# Autodesk Inventor assembly: Deck
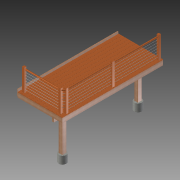
[picture p0: Inventor's stored thumbnail of the model, 180x180]
Saved by Autodesk Inventor 2015 (Build 190159000, 159)
## iProperties
Created: 2014-05-27
Part Number: Deck
Document SubType Name: Assembly
Designer: Haden
Mass: 751429 g
Surface Area: 376936 cm^2
Volume: 644413 cm^3
Density: 1.16607 g/cm^3
Author: Haden
## Documents named in this file (22)
- C:\Users\Haden\Desktop\Deck\Deck.iam
- C:\Users\Haden\Desktop\Deck\Footing.ipt
- C:\Users\Haden\Desktop\Deck\Ledger Board.ipt
- C:\Users\Haden\Desktop\Deck\Left End Board.ipt
- C:\Users\Haden\Desktop\Deck\Joist.ipt
- C:\Users\Haden\Desktop\Deck\Truss.ipt
- C:\Users\Haden\Desktop\Deck\TimberTech.ipt
- C:\Users\Haden\Desktop\Deck\Left Post.ipt
- C:\Users\Haden\Desktop\Deck\Right Post.ipt
- C:\Users\Haden\Desktop\Deck\TimberTech Post.ipt
- C:\Users\Haden\Desktop\Deck\Front Railing.ipt
- C:\Users\Haden\Desktop\Deck\Side Railing.ipt
- C:\Users\Haden\Desktop\Deck\Left Cable.ipt
- C:\Users\Haden\Desktop\Deck\Front Cable.ipt
- C:\Users\Haden\Desktop\Deck\corner cable.ipt
- C:\Users\Haden\Desktop\Deck\Corner Railing.ipt
- C:\Users\Haden\Desktop\Deck\Deck\AIP\FEA\b2f62dg5c.fins
- C:\Users\Haden\Desktop\Deck\Deck\AIP\FEA\b2f62dg5c.fsat
- C:\Users\Haden\Desktop\Deck\Deck\AIP\FEA\b2f62dg5c.ftes
- C:\Users\Haden\Desktop\Deck\Deck\AIP\FEA\b2f62dg5c.fwiz
- C:\Users\Haden\Desktop\Deck\Deck\AIP\FEA\b2f62dh28.fmsh
- C:\Users\Haden\Desktop\Deck\Deck\AIP\FEA\b2f62dh29.fres
## Components (49 placed, 15 different names)
1. Ledger Board:1 — Mate:1, Mate:3, Flush:2, Mate:7, Mate:8, Mate:9, Mate:10, Mate:11, Mate:12, Mate:13, Mate:14, Mate:15, Mate:16, Mate:17, Mate:18, Mate:19, Flush:55, Mate:21, Flush:65, Mate:51
2. Left End Board:1 — Mate:1, Flush:65, Flush:1, Flush:6, Mate:6, Flush:7, Flush:8, Mate:37, Mate:38
3. Truss:1 — Mate:4, Flush:4, Flush:5
4. Truss:2 — Mate:4, Flush:4, Flush:5, Flush:6, Mate:5, Mate:37, Mate:39, Flush:69, Flush:70
5. Truss:3 — Mate:6, Flush:7, Flush:8, Flush:78, Mate:47
6. Joist:1 — Mate:3, Flush:1, Flush:2, Mate:38, Mate:5, Flush:9, Flush:22, Mate:20, Mate:48
7. Joist:2 — Flush:9, Flush:10, Flush:22, Flush:23, Mate:7
8. Joist:3 — Flush:10, Flush:11, Flush:23, Flush:24, Mate:8
9. Joist:4 — Flush:11, Flush:12, Flush:24, Flush:25, Mate:9
10. Joist:5 — Flush:12, Flush:13, Flush:25, Flush:26, Mate:10
11. Joist:6 — Flush:13, Flush:14, Flush:26, Flush:27, Mate:11
12. Joist:7 — Flush:14, Flush:15, Flush:27, Flush:28, Mate:12
13. Joist:8 — Flush:15, Flush:16, Flush:28, Flush:29, Mate:13
14. Joist:9 — Flush:16, Flush:17, Flush:29, Flush:30, Mate:14
15. Joist:10 — Flush:17, Flush:18, Flush:30, Flush:31, Mate:15
16. Joist:11 — Flush:18, Flush:19, Flush:31, Flush:32, Mate:16
17. Joist:12 — Flush:19, Flush:20, Flush:32, Flush:33, Mate:17
18. Joist:13 — Flush:20, Flush:21, Flush:33, Flush:34, Mate:18
19. Joist:14 — Flush:21, Flush:34, Mate:19
20. TimberTech:1 — Flush:35, Flush:45, Mate:20, Flush:55, Mate:21, Mate:22
21. TimberTech:2 — Flush:35, Flush:36, Flush:45, Flush:46, Mate:22, Mate:23, Mate:61
22. TimberTech:3 — Flush:36, Flush:37, Flush:46, Flush:47, Mate:23, Mate:24
23. TimberTech:4 — Flush:37, Flush:38, Flush:47, Flush:48, Mate:24, Mate:25
24. TimberTech:5 — Flush:38, Flush:39, Flush:48, Flush:49, Mate:25, Mate:26
25. TimberTech:6 — Flush:39, Flush:40, Flush:49, Flush:50, Mate:26, Mate:27
26. TimberTech:7 — Flush:40, Flush:41, Flush:50, Flush:51, Mate:27, Mate:28
27. TimberTech:8 — Flush:41, Flush:42, Flush:51, Flush:52, Mate:28, Mate:29
28. TimberTech:9 — Flush:42, Flush:43, Flush:52, Flush:53, Mate:29, Mate:30
29. TimberTech:10 — Flush:43, Flush:44, Flush:53, Flush:54, Mate:30, Mate:31
30. TimberTech:11 — Flush:44, Flush:54, Mate:31, Flush:56, Flush:57, Mate:32
31. TimberTech:12 — Flush:56, Flush:57, Mate:32, Mate:68, Mate:71, Flush:86, Flush:87, Mate:74
32. TimberTech:13 — Flush:86, Flush:87, Mate:74
33. Footing:1 — Mate:40, Rotation:1, Rotation:2, Mate:43
34. Footing:2 — Mate:41, Rotation:1, Mate:42
35. Left Post:1 — Flush:66, Flush:67, Mate:39, Mate:40, Rotation:2, Mate:43, Flush:68, Flush:69, Flush:70
36. Right Post:1 — Flush:66, Flush:67, Mate:41, Mate:42, Flush:68
37. TimberTech Post:1 — Flush:71, Flush:74, Mate:49, Mate:50, Flush:80, Mate:55, Mate:70, Mate:73
38. TimberTech Post:2 — Flush:71, Flush:74, Flush:75, Mate:48, Mate:51, Mate:52, Flush:83, Mate:58
39. TimberTech Post:3 — Flush:75, Flush:76, Mate:45, Flush:78, Flush:79, Mate:47, Mate:49, Mate:50, Mate:53, Mate:57, Flush:84, Mate:62, Mate:69, Mate:72
40. TimberTech Post:4 — Flush:73, Flush:76, Flush:77, Mate:44, Mate:45, Flush:79, Mate:54, Mate:63
41. TimberTech Post:5 — Flush:73, Flush:77, Mate:44
42. Front Railing:1 — Mate:53, Flush:81, Flush:82, Mate:56, Mate:57
43. Front Railing:2 — Mate:54, Flush:82, Mate:56
44. Side Railing:1 — Mate:52, Flush:80, Mate:55, Flush:81, Flush:85
45. Left Cable:1 — Mate:58, Mate:59, Mate:60, Mate:61
46. Front Cable:1 — Mate:62, Mate:64, Mate:67
47. Front Cable:2 — Mate:63, Mate:64, Mate:65, Mate:66, Mate:67, Mate:68
48. corner cable:1 — Mate:69, Mate:70, Mate:71
49. Corner Railing:1 — Mate:72, Mate:73, Flush:85
## Relationships (148: Flush 78, Mate 68, RelateRotation 2)
- Mate:1: Ledger Board:1 ↔ Left End Board:1
- Flush:65: Ledger Board:1 ↔ Left End Board:1
- Mate:3: Ledger Board:1 ↔ Joist:1
- Flush:1: Left End Board:1 ↔ Joist:1
- Flush:2: Ledger Board:1 ↔ Joist:1
- Mate:38: Left End Board:1 ↔ Joist:1
- Mate:4: Truss:1 ↔ Truss:2
- Flush:4: Truss:1 ↔ Truss:2
- Flush:5: Truss:1 ↔ Truss:2
- Flush:6: Left End Board:1 ↔ Truss:2
- Mate:5: Truss:2 ↔ Joist:1
- Mate:6: Left End Board:1 ↔ Truss:3
- Flush:7: Left End Board:1 ↔ Truss:3
- Flush:8: Left End Board:1 ↔ Truss:3
- Flush:9 (304.8 mm): Joist:1 ↔ Joist:2
- Flush:10 (304.8 mm): Joist:2 ↔ Joist:3
- Flush:11 (304.8 mm): Joist:3 ↔ Joist:4
- Flush:12 (304.8 mm): Joist:4 ↔ Joist:5
- Flush:13 (304.8 mm): Joist:5 ↔ Joist:6
- Flush:14 (304.8 mm): Joist:6 ↔ Joist:7
- Flush:15 (304.8 mm): Joist:7 ↔ Joist:8
- Flush:16 (304.8 mm): Joist:8 ↔ Joist:9
- Flush:17 (304.8 mm): Joist:9 ↔ Joist:10
- Flush:18 (304.8 mm): Joist:10 ↔ Joist:11
- Flush:19 (304.8 mm): Joist:11 ↔ Joist:12
- Flush:20 (304.8 mm): Joist:12 ↔ Joist:13
- Flush:21 (304.8 mm): Joist:13 ↔ Joist:14
- Flush:22: Joist:1 ↔ Joist:2
- Flush:23: Joist:2 ↔ Joist:3
- Flush:24: Joist:3 ↔ Joist:4
- Flush:25: Joist:4 ↔ Joist:5
- Flush:26: Joist:5 ↔ Joist:6
- Flush:27: Joist:6 ↔ Joist:7
- Flush:28: Joist:7 ↔ Joist:8
- Flush:29: Joist:8 ↔ Joist:9
- Flush:30: Joist:9 ↔ Joist:10
- Flush:31: Joist:10 ↔ Joist:11
- Flush:32: Joist:11 ↔ Joist:12
- Flush:33: Joist:12 ↔ Joist:13
- Flush:34: Joist:13 ↔ Joist:14
- Mate:7: Ledger Board:1 ↔ Joist:2
- Mate:8: Ledger Board:1 ↔ Joist:3
- Mate:9: Ledger Board:1 ↔ Joist:4
- Mate:10: Ledger Board:1 ↔ Joist:5
- Mate:11: Ledger Board:1 ↔ Joist:6
- Mate:12: Ledger Board:1 ↔ Joist:7
- Mate:13: Ledger Board:1 ↔ Joist:8
- Mate:14: Ledger Board:1 ↔ Joist:9
- Mate:15: Ledger Board:1 ↔ Joist:10
- Mate:16: Ledger Board:1 ↔ Joist:11
- Mate:17: Ledger Board:1 ↔ Joist:12
- Mate:18: Ledger Board:1 ↔ Joist:13
- Mate:19: Ledger Board:1 ↔ Joist:14
- Flush:35: TimberTech:1 ↔ TimberTech:2
- Flush:36: TimberTech:2 ↔ TimberTech:3
- Flush:37: TimberTech:3 ↔ TimberTech:4
- Flush:38: TimberTech:4 ↔ TimberTech:5
- Flush:39: TimberTech:5 ↔ TimberTech:6
- Flush:40: TimberTech:6 ↔ TimberTech:7
- Flush:41: TimberTech:7 ↔ TimberTech:8
- Flush:42: TimberTech:8 ↔ TimberTech:9
- Flush:43: TimberTech:9 ↔ TimberTech:10
- Flush:44: TimberTech:10 ↔ TimberTech:11
- Flush:45: TimberTech:1 ↔ TimberTech:2
- Flush:46: TimberTech:2 ↔ TimberTech:3
- Flush:47: TimberTech:3 ↔ TimberTech:4
- Flush:48: TimberTech:4 ↔ TimberTech:5
- Flush:49: TimberTech:5 ↔ TimberTech:6
- Flush:50: TimberTech:6 ↔ TimberTech:7
- Flush:51: TimberTech:7 ↔ TimberTech:8
- Flush:52: TimberTech:8 ↔ TimberTech:9
- Flush:53: TimberTech:9 ↔ TimberTech:10
- Flush:54: TimberTech:10 ↔ TimberTech:11
- Mate:20: Joist:1 ↔ TimberTech:1
- Flush:55: Ledger Board:1 ↔ TimberTech:1
- Mate:21 (2.54 mm): Ledger Board:1 ↔ TimberTech:1
- Mate:22 (2.54 mm): TimberTech:1 ↔ TimberTech:2
- Mate:23 (2.54 mm): TimberTech:2 ↔ TimberTech:3
- Mate:24 (2.54 mm): TimberTech:3 ↔ TimberTech:4
- Mate:25 (2.54 mm): TimberTech:4 ↔ TimberTech:5
- Mate:26 (2.54 mm): TimberTech:5 ↔ TimberTech:6
- Mate:27 (2.54 mm): TimberTech:6 ↔ TimberTech:7
- Mate:28 (2.54 mm): TimberTech:7 ↔ TimberTech:8
- Mate:29 (2.54 mm): TimberTech:8 ↔ TimberTech:9
- Mate:30 (2.54 mm): TimberTech:9 ↔ TimberTech:10
- Mate:31 (2.54 mm): TimberTech:10 ↔ TimberTech:11
- Flush:56: TimberTech:11 ↔ TimberTech:12
- Flush:57: TimberTech:11 ↔ TimberTech:12
- Mate:32 (2.54 mm): TimberTech:11 ↔ TimberTech:12
- Mate:37: Left End Board:1 ↔ Truss:2
- Flush:66: Left Post:1 ↔ Right Post:1
- Flush:67: Left Post:1 ↔ Right Post:1
- Mate:39: Truss:2 ↔ Left Post:1
- Mate:40: Footing:1 ↔ Left Post:1
- Mate:41: Footing:2 ↔ Right Post:1
- Rotation:1 [RelateRotation] (1 ul): Footing:1 ↔ Footing:2
- Rotation:2 [RelateRotation] (1 ul): Footing:1 ↔ Left Post:1
- Mate:42: Footing:2 ↔ Right Post:1
- Mate:43: Footing:1 ↔ Left Post:1
- Flush:68 (3048 mm): Left Post:1 ↔ Right Post:1
- Flush:69 (304.8 mm): Truss:2 ↔ Left Post:1
- Flush:70 (38.1 mm): Truss:2 ↔ Left Post:1
- Flush:71: TimberTech Post:1 ↔ TimberTech Post:2
- Flush:73: TimberTech Post:4 ↔ TimberTech Post:5
- Flush:74: TimberTech Post:1 ↔ TimberTech Post:2
- Flush:75: TimberTech Post:2 ↔ TimberTech Post:3
- Flush:76: TimberTech Post:3 ↔ TimberTech Post:4
- Flush:77: TimberTech Post:4 ↔ TimberTech Post:5
- Mate:44 (1778 mm): TimberTech Post:4 ↔ TimberTech Post:5
- Mate:45 (1778 mm): TimberTech Post:3 ↔ TimberTech Post:4
- Flush:78: Truss:3 ↔ TimberTech Post:3
- Flush:79: TimberTech Post:3 ↔ TimberTech Post:4
- Mate:47: Truss:3 ↔ TimberTech Post:3
- Mate:48: Joist:1 ↔ TimberTech Post:2
- Mate:49 (25.4 mm): TimberTech Post:1 ↔ TimberTech Post:3
- Mate:50 (25.4 mm): TimberTech Post:1 ↔ TimberTech Post:3
- Mate:51 (95.504 mm): Ledger Board:1 ↔ TimberTech Post:2
- Mate:52: TimberTech Post:2 ↔ Side Railing:1
- Mate:53: TimberTech Post:3 ↔ Front Railing:1
- Mate:54: TimberTech Post:4 ↔ Front Railing:2
- Flush:80 (50.8 mm): TimberTech Post:1 ↔ Side Railing:1
- Mate:55 (-44.45 mm): TimberTech Post:1 ↔ Side Railing:1
- Flush:81: Front Railing:1 ↔ Side Railing:1
- Flush:82: Front Railing:1 ↔ Front Railing:2
- Mate:56: Front Railing:1 ↔ Front Railing:2
- Mate:57 (-44.45 mm): TimberTech Post:3 ↔ Front Railing:1
- Flush:83 (-44.45 mm): TimberTech Post:2
- Mate:58: TimberTech Post:2 ↔ Left Cable:1
- Mate:59: Left Cable:1
- Mate:60: Left Cable:1
- Mate:61 (101.6 mm): TimberTech:2 ↔ Left Cable:1
- Flush:84 (-44.45 mm): TimberTech Post:3
- Mate:62: TimberTech Post:3 ↔ Front Cable:1
- Mate:63: TimberTech Post:4 ↔ Front Cable:2
- Mate:64: Front Cable:1 ↔ Front Cable:2
- Mate:65: Front Cable:2
- Mate:66: Front Cable:2
- Mate:67: Front Cable:1 ↔ Front Cable:2
- Mate:68 (101.6 mm): TimberTech:12 ↔ Front Cable:2
- Mate:69: TimberTech Post:3 ↔ corner cable:1
- Mate:70: TimberTech Post:1 ↔ corner cable:1
- Mate:71 (101.6 mm): TimberTech:12 ↔ corner cable:1
- Mate:72: TimberTech Post:3 ↔ Corner Railing:1
- Mate:73: TimberTech Post:1 ↔ Corner Railing:1
- Flush:85: Side Railing:1 ↔ Corner Railing:1
- Flush:86: TimberTech:12 ↔ TimberTech:13
- Flush:87: TimberTech:12 ↔ TimberTech:13
- Mate:74 (2.54 mm): TimberTech:12 ↔ TimberTech:13
